# Autodesk Inventor assembly: Модуль перемещения
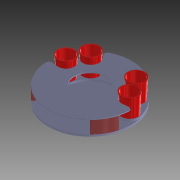
[picture p0: Inventor's stored thumbnail of the model, 180x180]
Saved by Autodesk Inventor 2022 (Build 260153000, 153)
## iProperties
Created: 2025-01-11
Part Number: Модуль перемещения
Document SubType Name: Assembly
Designer: Ivan
Mass: 676.614 g
Surface Area: 3324.37 cm^2
Volume: 676.614 cm^3
Density: 1 g/cm^3
Author: Ivan
Title: Модуль перемещения
## Documents named in this file (6)
- E:\Предпроф 2025\Shoter_1_ZIP\Модуль перемещения.iam
- E:\Предпроф 2025\Shoter_1_ZIP\Диск_фиксирующий.ipt
- E:\Предпроф 2025\Shoter_1_ZIP\Диск опорный.ipt
- E:\Предпроф 2025\Shoter_1_ZIP\Диск_фиксатор.ipt
- E:\Предпроф 2025\Shoter_1_ZIP\Стойка.ipt
- E:\Предпроф 2025\Shoter_1_ZIP\Стакан_В2.ipt
## Components (10 placed, 5 different names)
1. Диск_фиксатор:1 — Совмещение:3, Совмещение:4, Заподлицо:11, Совмещение:12, Совмещение:13, Совмещение:14
2. Диск_фиксирующий:2 — Совмещение:7, Совмещение:8, Совмещение:9, Совмещение:10
3. Диск опорный:2 — Совмещение:1, Совмещение:2, Заподлицо:1, Совмещение:3, Совмещение:4, Совмещение:5, Совмещение:6, Совмещение:7, Совмещение:8, Совмещение:11, Совмещение:15, Совмещение:16, Совмещение:17
4. Стакан_В2:2 — Совмещение:10, Совмещение:11
5. Стакан_В2:3 — Совмещение:14, Совмещение:15
6. Стакан_В2:4 — Совмещение:13, Совмещение:16
7. Стакан_В2:5 — Совмещение:12, Совмещение:17
8. Стойка:1 — Совмещение:5, Совмещение:6, Совмещение:9
9. Стойка:2
10. Стойка:3
## Component patterns: (3 elements, first: Стойка:1)
## Relationships (19: Mate 17, Flush 2)
- Совмещение:1 [Mate]: Диск опорный:2
- Совмещение:2 [Mate]: Диск опорный:2
- Заподлицо:1 [Flush]: Диск опорный:2
- Совмещение:3 [Mate]: Диск_фиксатор:1 ↔ Диск опорный:2
- Совмещение:4 [Mate]: Диск_фиксатор:1 ↔ Диск опорный:2
- Совмещение:5 [Mate]: Диск опорный:2 ↔ Стойка:1
- Совмещение:6 [Mate]: Диск опорный:2 ↔ Стойка:1
- Совмещение:7 [Mate]: Диск_фиксирующий:2 ↔ Диск опорный:2
- Совмещение:8 [Mate]: Диск_фиксирующий:2 ↔ Диск опорный:2
- Совмещение:9 [Mate]: Диск_фиксирующий:2 ↔ Стойка:1
- Заподлицо:11 [Flush]: Диск_фиксатор:1
- Совмещение:10 [Mate]: Диск_фиксирующий:2 ↔ Стакан_В2:2
- Совмещение:11 [Mate]: Диск опорный:2 ↔ Стакан_В2:2
- Совмещение:12 [Mate]: Диск_фиксатор:1 ↔ Стакан_В2:5
- Совмещение:13 [Mate]: Диск_фиксатор:1 ↔ Стакан_В2:4
- Совмещение:14 [Mate]: Диск_фиксатор:1 ↔ Стакан_В2:3
- Совмещение:15 [Mate]: Диск опорный:2 ↔ Стакан_В2:3
- Совмещение:16 [Mate]: Диск опорный:2 ↔ Стакан_В2:4
- Совмещение:17 [Mate]: Диск опорный:2 ↔ Стакан_В2:5
